# Autodesk Inventor assembly: total_model
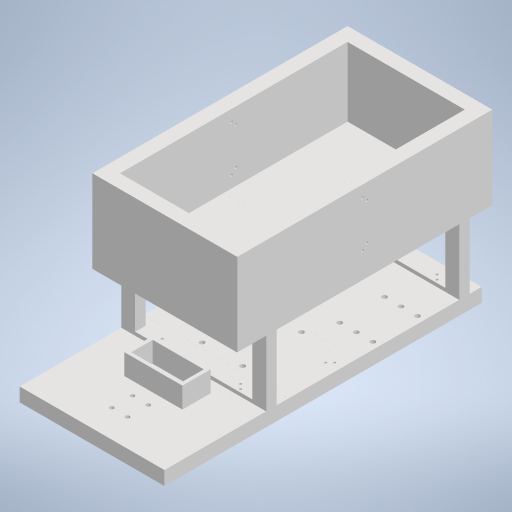
[picture p0: Inventor's stored thumbnail of the model, 512x512]
Saved by Autodesk Inventor 2023 (Build 270158000, 158)
## iProperties
Created: 2022-10-28
Part Number: total_model
Document SubType Name: Assembly
Designer: inigo
Author: inigo
## Documents named in this file (6)
- C:\Users\papel\FoBo\model\total_model.iam
- C:\Users\papel\FoBo\model\base_front.ipt
- C:\Users\papel\FoBo\model\base_mid.ipt
- C:\Users\papel\FoBo\model\base_back.ipt
- C:\Users\papel\FoBo\model\container_front.ipt
- C:\Users\papel\FoBo\model\container_back.ipt
## Components (5 placed, 5 different names)
1. base_front:1 — Coincidencia:1, Coincidencia:2, Coincidencia:3
2. base_mid:1 — Coincidencia:1, Coincidencia:2, Coincidencia:3, Coincidencia:4, Coincidencia:5, Coincidencia:6
3. base_back:1 — Coincidencia:4, Coincidencia:5, Coincidencia:6, Coincidencia:9, Nivelación:3, Coincidencia:10
4. container_front:1 — Nivelación:1, Coincidencia:7, Coincidencia:8, Nivelación:2
5. container_back:1 — Nivelación:1, Coincidencia:7, Coincidencia:8, Nivelación:2, Coincidencia:9, Nivelación:3, Coincidencia:10
## Relationships (13: Mate 10, Flush 3)
- Coincidencia:1 [Mate]: base_front:1 ↔ base_mid:1
- Coincidencia:2 [Mate]: base_front:1 ↔ base_mid:1
- Coincidencia:3 [Mate]: base_front:1 ↔ base_mid:1
- Coincidencia:4 [Mate]: base_mid:1 ↔ base_back:1
- Coincidencia:5 [Mate]: base_mid:1 ↔ base_back:1
- Coincidencia:6 [Mate]: base_mid:1 ↔ base_back:1
- Nivelación:1 [Flush]: container_front:1 ↔ container_back:1
- Coincidencia:7 [Mate]: container_front:1 ↔ container_back:1
- Coincidencia:8 [Mate]: container_front:1 ↔ container_back:1
- Nivelación:2 [Flush]: container_front:1 ↔ container_back:1
- Coincidencia:9 [Mate]: base_back:1 ↔ container_back:1
- Nivelación:3 [Flush]: base_back:1 ↔ container_back:1
- Coincidencia:10 [Mate]: base_back:1 ↔ container_back:1
